# Autodesk Inventor assembly: FemaleHeaderPin_1x3
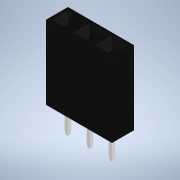
[picture p0: Inventor's stored thumbnail of the model, 180x180]
Saved by Autodesk Inventor 2021 (Build 250183000, 183)
## iProperties
Created: 2020-01-02
Part Number: FemaleHeaderPin_1x3
Document SubType Name: Assembly
Designer: ermoz
Mass: 0.213921 g
Surface Area: 4.48219 cm^2
Volume: 0.213921 cm^3
Density: 1 g/cm^3
Author: ermoz
## Documents named in this file (2)
- D:\Moje Wyczyny\My_Poor_Projects\Sneak100_MiniSumo\minisumo-sneak100\mechanics\ElectricElements\FemaleHeaderPin_1x3.iam
- D:\Moje Wyczyny\My_Poor_Projects\Sneak100_MiniSumo\minisumo-sneak100\mechanics\ElectricElements\FemaleHederPin.ipt
## Components (3 placed, 1 different names)
1. FemaleHederPin:1 — Mate:1, Flush:1, Flush:7
2. FemaleHederPin:2 — Mate:1, Mate:2, Flush:1, Flush:2, Flush:7, Flush:8
3. FemaleHederPin:3 — Mate:2, Flush:2, Flush:8
## Relationships (6: Flush 4, Mate 2)
- Mate:1: FemaleHederPin:1 ↔ FemaleHederPin:2
- Mate:2: FemaleHederPin:2 ↔ FemaleHederPin:3
- Flush:1: FemaleHederPin:1 ↔ FemaleHederPin:2
- Flush:2: FemaleHederPin:2 ↔ FemaleHederPin:3
- Flush:7: FemaleHederPin:1 ↔ FemaleHederPin:2
- Flush:8: FemaleHederPin:2 ↔ FemaleHederPin:3
